# Autodesk Inventor assembly: Assembly
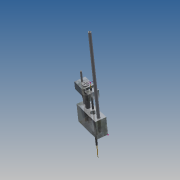
[picture p0: Inventor's stored thumbnail of the model, 180x180]
Saved by Autodesk Inventor 2020 (Build 240168000, 168)
## iProperties
Created: 2019-02-08
Part Number: Assembly
Material: 일반
Document SubType Name: Assembly
Designer: Knowblesse
Author: Knowblesse
Revision Number: 1.0
## Documents named in this file (10)
- C:\VCF\Microdrive\Assembly.iam
- C:\VCF\Microdrive\Bot.ipt
- C:\VCF\Microdrive\Top.ipt
- C:\VCF\Microdrive\19G_Stage.ipt
- C:\VCF\Microdrive\23G_Holder.ipt
- C:\VCF\Microdrive\23G_Pillar.ipt
- C:\VCF\Microdrive\Nut.ipt
- C:\VCF\Microdrive\Polyimide.ipt
- C:\VCF\Microdrive\Screw.ipt
- C:\VCF\Microdrive\Tetrode.ipt
## Components (9 placed, 9 different names)
1. Bot:1 — 회전:3, 원통형:4, 강체:6
2. Top:1 — 회전:1, 회전:2, 원통형:3, 강체:5
3. 19G_Stage:1 — 회전:3
4. 23G_Holder:1 — 원통형:3, 강체:6
5. 23G_Pillar:1 — 강체:3, 강체:5, 원통형:4
6. Nut:1 — 회전:2
7. Polyimide:1 — 강체:3, 강체:4
8. Screw:1 — 회전:1
9. Tetrode:1 — 강체:4
## Relationships (9: WeldJoint 4, RevoluteJoint 3, CylindricalJoint 2)
- 회전:1 [RevoluteJoint]: Top:1 ↔ Screw:1
- 회전:2 [RevoluteJoint]: Top:1 ↔ Nut:1
- 원통형:3 [CylindricalJoint]: Top:1 ↔ 23G_Holder:1
- 강체:3 [WeldJoint] (-1 mm): 23G_Pillar:1 ↔ Polyimide:1
- 강체:4 [WeldJoint] (1 mm): Polyimide:1 ↔ Tetrode:1
- 회전:3 [RevoluteJoint]: Bot:1 ↔ 19G_Stage:1
- 강체:5 [WeldJoint] (1 mm): Top:1 ↔ 23G_Pillar:1
- 원통형:4 [CylindricalJoint]: Bot:1 ↔ 23G_Pillar:1
- 강체:6 [WeldJoint]: Bot:1 ↔ 23G_Holder:1
